# Autodesk Inventor assembly: avionics box
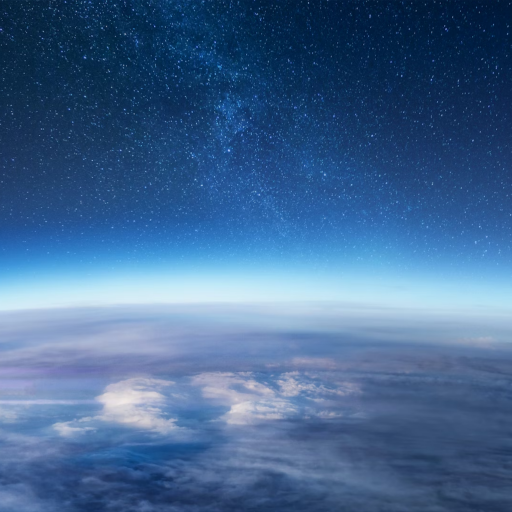
[picture p0: Inventor's stored thumbnail of the model, 512x512]
Saved by Autodesk Inventor 2023 (Build 270158000, 158)
## iProperties
Created: 2023-03-23
Part Number: avionics box
Document SubType Name: Assembly
Designer: 310611102
Mass: 302.953 g
Surface Area: 1971.44 cm^2
Volume: 120.675 cm^3
Density: 2.51049 g/cm^3
Author: 310611102
## Documents named in this file (15)
- C:\Users\310611102\Documents\Inventor\SSR\avionics_2023ver\electronics\avionics box.iam
- C:\Users\310611102\Documents\Inventor\SSR\avionics_2023ver\electronics\STM32 Communication Board ver1.0.ipt
- C:\Users\310611102\Documents\Inventor\SSR\avionics_2023ver\electronics\Power supply board.ipt
- C:\Users\310611102\Documents\Inventor\SSR\avionics_2023ver\electronics\copper_pillar_M3_L15.ipt
- C:\Users\310611102\Documents\Inventor\SSR\avionics_2023ver\electronics\MTI-7\MTi 1-series v3.iam
- C:\Users\310611102\Documents\Inventor\SSR\avionics_2023ver\electronics\LoRa_board.ipt
- C:\Users\310611102\Documents\Inventor\SSR\avionics_2023ver\electronics\empty_board.ipt
- C:\Users\310611102\Documents\Inventor\SSR\avionics_2023ver\electronics\copper_pillar_M3_L25.ipt
- C:\Users\310611102\Documents\Inventor\SSR\avionics_2023ver\electronics\shield box\shieldbox_ver2\PCB_board_box.iam
- C:\Users\310611102\Documents\Inventor\SSR\avionics_2023ver\electronics\washerM3x0.5h.ipt
- C:\Users\310611102\Documents\Inventor\SSR\avionics_2023ver\electronics\copper_pillar_M3_L4.ipt
- C:\Users\310611102\Documents\Inventor\SSR\avionics_2023ver\electronics\cooling_fin.ipt
- C:\Users\310611102\Documents\Inventor\SSR\avionics_2023ver\electronics\cooling_fan.ipt
- C:\Users\310611102\Documents\Inventor\Content Center Files\R2023\en-US\ISO 4762(2)\ISO 4762 - M4 x 16ISO.ipt
- C:\Users\310611102\Documents\Inventor\Content Center Files\R2023\en-US\ISO 4032(2)\ISO 4032 - M4 - ISO.ipt
## Components (52 placed, 14 different names)
1. STM32 Communication Board ver1.0:1 — Insert:52, Insert:53, Insert:54, Insert:55, Insert:56, Insert:57, Mate:15
2. Power supply board:1 — Mate:3, Mate:4, Mate:5, Insert:36, Insert:37, Insert:38, Insert:39, Insert:44, Insert:45, Insert:46, Insert:47
3. copper_pillar_M3_L15:1 — Insert:42, Insert:50
4. copper_pillar_M3_L15:3 — Insert:40, Insert:49
5. MTi 1-series v3:1 [sub-assembly] — Insert:8, Insert:9, Insert:35
6. LoRa_board:1 — Mate:3, Mate:4, Mate:5
7. empty_board:1 — Insert:8, Insert:9, Insert:35, Cylindrical:1, Cylindrical:2
8. copper_pillar_M3_L25:1 — Insert:60, Insert:75, Cylindrical:2
9. copper_pillar_M3_L25:2 — Insert:62, Insert:76, Cylindrical:1
10. copper_pillar_M3_L25:3 — Insert:59, Insert:61, Insert:74
11. copper_pillar_M3_L25:4 — Insert:58, Insert:73
12. copper_pillar_M3_L15:13 — Insert:43, Insert:51
13. copper_pillar_M3_L15:14 — Insert:41, Insert:48
14. PCB_board_box:1 [sub-assembly] — Mate:9, Mate:10, Insert:71, Insert:72, Insert:77, Insert:78, Mate:17, Insert:83, Insert:84, Insert:85
15. washerM3x0.5h:1 — Insert:36, Insert:42
16. washerM3x0.5h:2 — Insert:37, Insert:43
17. washerM3x0.5h:3 — Insert:38, Insert:40
18. washerM3x0.5h:4 — Insert:39, Insert:41
19. washerM3x0.5h:5 — Insert:45, Insert:65
20. washerM3x0.5h:6 — Insert:44, Insert:66
21. washerM3x0.5h:7 — Insert:46, Insert:63
22. washerM3x0.5h:8 — Insert:47, Insert:64
23. washerM3x0.5h:9 — Insert:48
24. washerM3x0.5h:10 — Insert:49
25. washerM3x0.5h:11 — Insert:50, Insert:53
26. washerM3x0.5h:12 — Insert:51, Insert:52
27. washerM3x0.5h:13 — Insert:57, Insert:59, Insert:61
28. washerM3x0.5h:14 — Insert:56, Insert:58
29. washerM3x0.5h:15 — Insert:55, Insert:62
30. washerM3x0.5h:16 — Insert:54, Insert:60
31. copper_pillar_M3_L4:1 — Insert:63, Insert:69
32. copper_pillar_M3_L4:2 — Insert:66, Insert:68
33. copper_pillar_M3_L4:3 — Insert:65, Insert:70
34. copper_pillar_M3_L4:4 — Insert:64, Insert:67
35. washerM3x0.5h:17 — Insert:67, Insert:72
36. washerM3x0.5h:18 — Insert:69
37. washerM3x0.5h:19 — Insert:68
38. washerM3x0.5h:20 — Insert:70, Insert:71
39. washerM3x0.5h:21 — Insert:73
40. washerM3x0.5h:22 — Insert:75
41. washerM3x0.5h:23 — Insert:74
42. washerM3x0.5h:24 — Insert:76
43. cooling_fin:1 — Mate:15
44. cooling_fan:1 — Insert:77, Insert:78, Insert:79, Insert:80, Insert:81, Insert:82
45. ISO 4762 M4 x 16:1 — Insert:79, Mate:16
46. ISO 4762 M4 x 16:2 — Insert:80
47. ISO 4762 M4 x 16:3 — Insert:81
48. ISO 4762 M4 x 16:4 — Insert:82
49. ISO 4032 M4:1 — Mate:16, Mate:17
50. ISO 4032 M4:2 — Insert:83
51. ISO 4032 M4:3 — Insert:84
52. ISO 4032 M4:4 — Insert:85
## Relationships (64: Insert 53, Mate 9, CylindricalJoint 2)
- Mate:3: Power supply board:1 ↔ LoRa_board:1
- Mate:4: Power supply board:1 ↔ LoRa_board:1
- Mate:5: Power supply board:1 ↔ LoRa_board:1
- Insert:8: MTi 1-series v3:1 ↔ empty_board:1
- Insert:9: MTi 1-series v3:1 ↔ empty_board:1
- Insert:35: MTi 1-series v3:1 ↔ empty_board:1
- Mate:9: PCB_board_box:1
- Mate:10: PCB_board_box:1
- Mate:14
- Insert:36: Power supply board:1 ↔ washerM3x0.5h:1
- Insert:37: Power supply board:1 ↔ washerM3x0.5h:2
- Insert:38: Power supply board:1 ↔ washerM3x0.5h:3
- Insert:39: Power supply board:1 ↔ washerM3x0.5h:4
- Insert:40: copper_pillar_M3_L15:3 ↔ washerM3x0.5h:3
- Insert:41: copper_pillar_M3_L15:14 ↔ washerM3x0.5h:4
- Insert:42: copper_pillar_M3_L15:1 ↔ washerM3x0.5h:1
- Insert:43: copper_pillar_M3_L15:13 ↔ washerM3x0.5h:2
- Insert:44: Power supply board:1 ↔ washerM3x0.5h:6
- Insert:45: Power supply board:1 ↔ washerM3x0.5h:5
- Insert:46: Power supply board:1 ↔ washerM3x0.5h:7
- Insert:47: Power supply board:1 ↔ washerM3x0.5h:8
- Insert:48: copper_pillar_M3_L15:14 ↔ washerM3x0.5h:9
- Insert:49: copper_pillar_M3_L15:3 ↔ washerM3x0.5h:10
- Insert:50: copper_pillar_M3_L15:1 ↔ washerM3x0.5h:11
- Insert:51: copper_pillar_M3_L15:13 ↔ washerM3x0.5h:12
- Insert:52: STM32 Communication Board ver1.0:1 ↔ washerM3x0.5h:12
- Insert:53: STM32 Communication Board ver1.0:1 ↔ washerM3x0.5h:11
- Insert:54: STM32 Communication Board ver1.0:1 ↔ washerM3x0.5h:16
- Insert:55: STM32 Communication Board ver1.0:1 ↔ washerM3x0.5h:15
- Insert:56: STM32 Communication Board ver1.0:1 ↔ washerM3x0.5h:14
- Insert:57: STM32 Communication Board ver1.0:1 ↔ washerM3x0.5h:13
- Insert:58: copper_pillar_M3_L25:4 ↔ washerM3x0.5h:14
- Insert:59: copper_pillar_M3_L25:3 ↔ washerM3x0.5h:13
- Insert:60: copper_pillar_M3_L25:1 ↔ washerM3x0.5h:16
- Insert:61: copper_pillar_M3_L25:3 ↔ washerM3x0.5h:13
- Insert:62: copper_pillar_M3_L25:2 ↔ washerM3x0.5h:15
- Insert:63: washerM3x0.5h:7 ↔ copper_pillar_M3_L4:1
- Insert:64: washerM3x0.5h:8 ↔ copper_pillar_M3_L4:4
- Insert:65: washerM3x0.5h:5 ↔ copper_pillar_M3_L4:3
- Insert:66: washerM3x0.5h:6 ↔ copper_pillar_M3_L4:2
- Insert:67: copper_pillar_M3_L4:4 ↔ washerM3x0.5h:17
- Insert:68: copper_pillar_M3_L4:2 ↔ washerM3x0.5h:19
- Insert:69: copper_pillar_M3_L4:1 ↔ washerM3x0.5h:18
- Insert:70: copper_pillar_M3_L4:3 ↔ washerM3x0.5h:20
- Insert:71: PCB_board_box:1 ↔ washerM3x0.5h:20
- Insert:72: PCB_board_box:1 ↔ washerM3x0.5h:17
- Insert:73: copper_pillar_M3_L25:4 ↔ washerM3x0.5h:21
- Insert:74: copper_pillar_M3_L25:3 ↔ washerM3x0.5h:23
- Insert:75: copper_pillar_M3_L25:1 ↔ washerM3x0.5h:22
- Insert:76: copper_pillar_M3_L25:2 ↔ washerM3x0.5h:24
- Cylindrical:1: empty_board:1 ↔ copper_pillar_M3_L25:2
- Cylindrical:2: empty_board:1 ↔ copper_pillar_M3_L25:1
- Mate:15: STM32 Communication Board ver1.0:1 ↔ cooling_fin:1
- Insert:77: PCB_board_box:1 ↔ cooling_fan:1
- Insert:78: PCB_board_box:1 ↔ cooling_fan:1
- Insert:79: cooling_fan:1 ↔ ISO 4762 M4 x 16:1
- Mate:16: ISO 4762 M4 x 16:1 ↔ ISO 4032 M4:1
- Mate:17: PCB_board_box:1 ↔ ISO 4032 M4:1
- Insert:80: cooling_fan:1 ↔ ISO 4762 M4 x 16:2
- Insert:81: cooling_fan:1 ↔ ISO 4762 M4 x 16:3
- Insert:82: cooling_fan:1 ↔ ISO 4762 M4 x 16:4
- Insert:83: PCB_board_box:1 ↔ ISO 4032 M4:2
- Insert:84: PCB_board_box:1 ↔ ISO 4032 M4:3
- Insert:85: PCB_board_box:1 ↔ ISO 4032 M4:4
